# Autodesk Inventor assembly: left pneumatics board
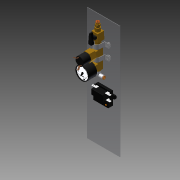
[picture p0: Inventor's stored thumbnail of the model, 180x180]
Saved by Autodesk Inventor 2014 SP1 (Build 180222100, 222)
## iProperties
Created: 2014-01-20
Part Number: left pneumatics board
Document SubType Name: Assembly
Designer: Arpan
Author: Arpan
## Documents named in this file (4)
- C:\Users\Arpan\Documents\GitHub\2014buildCAD\pneumatics board\left pneumatics board.iam
- C:\Users\Arpan\Documents\GitHub\2014buildCAD\pneumatics board\pneumatics board 1.ipt
- C:\Users\Arpan\Documents\GitHub\2014buildCAD\pneumatics board\pneumatic thing 1.iam
- C:\Users\Arpan\Documents\GitHub\2014buildCAD\electrical\CS_Relay_SPIKE-RELAY-H.ipt
## Components (3 placed, 3 different names)
1. pneumatics board 1:1 — Mate:1, Mate:2
2. pneumatic thing 1:1 [sub-assembly] — Mate:1
3. CS_Relay_SPIKE-RELAY-H:1 — Mate:2
## Relationships (2: Mate 2)
- Mate:1: pneumatics board 1:1 ↔ pneumatic thing 1:1
- Mate:2: pneumatics board 1:1 ↔ CS_Relay_SPIKE-RELAY-H:1
